# Autodesk Inventor assembly: Baugruppe1
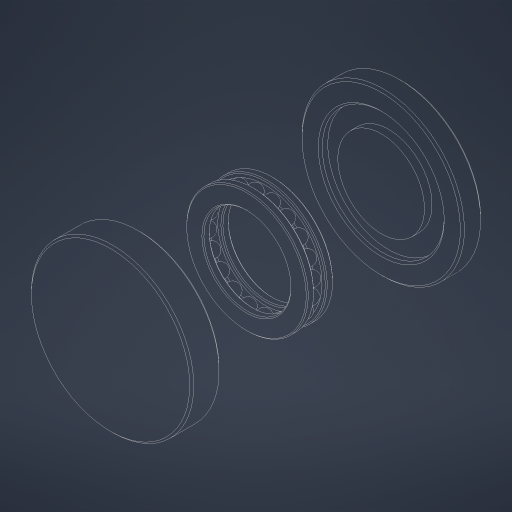
[picture p0: Inventor's stored thumbnail of the model, 512x512]
Saved by Autodesk Inventor 2024 (Build 280153000, 153)
## iProperties
Created: 2025-03-30
Part Number: Baugruppe1
Document SubType Name: Assembly
Designer: Simon
Author: Simon
## Documents named in this file (4)
- C:\Users\Simon\Desktop\Studium\4.Semester\Rapid Enginering\Baugruppe1.iam
- C:\Users\Simon\Desktop\Studium\4.Semester\Rapid Enginering\Bauteil1.ipt
- C:\Users\Simon\Desktop\Studium\4.Semester\Rapid Enginering\Spinner_bottom.ipt
- C:\Users\Simon\Desktop\Studium\4.Semester\Rapid Enginering\Spinner_top.ipt
## Components (3 placed, 3 different names)
1. Bauteil1:1 — Passend:1
2. Spinner_bottom:1 — Passend:1, Passend:2
3. Spinner_top:1 — Passend:2
## Relationships (2: Mate 2)
- Passend:1 [Mate]: Bauteil1:1 ↔ Spinner_bottom:1
- Passend:2 [Mate]: Spinner_bottom:1 ↔ Spinner_top:1
